# Autodesk Inventor assembly: Riser Base
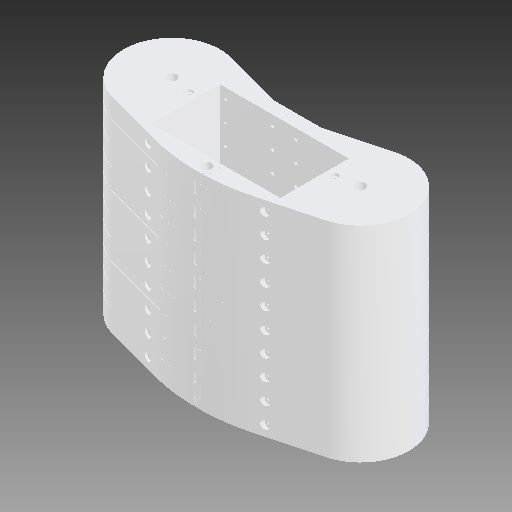
[picture p0: Inventor's stored thumbnail of the model, 512x512]
Saved by Autodesk Inventor 2017 SP1 (Build 210196100, 196)
## iProperties
Created: 2017-08-15
Part Number: Riser Base
Document SubType Name: Assembly
Designer: Zach
Author: Zach
## Documents named in this file (3)
- C:\Users\Zach\Documents\GitHub\cr-laundry-robot\src\Base\Rise Base Assembly\Riser Base.iam
- C:\Users\Zach\Documents\GitHub\cr-laundry-robot\src\Base\Rise Base Assembly\RB001.ipt
- C:\Users\Zach\Documents\GitHub\cr-laundry-robot\src\Base\Rise Base Assembly\RB002.ipt
## Components (40 placed, 2 different names)
1. RB001:1 — Mate:2, Mate:5, Mate:6, Mate:9, Mate:10, Mate:12, Mate:70
2. RB002:1 — Mate:1, Mate:9, Mate:10, Mate:69
3. RB001:2 — Mate:3, Mate:5, Mate:6, Mate:7, Mate:8, Mate:11, Mate:13
4. RB002:2 — Mate:4, Mate:7, Mate:8, Mate:68
5. RB001:3 — Mate:70, Mate:73
6. RB002:3 — Mate:69, Mate:72
7. RB001:4
8. RB002:4 — Mate:68, Mate:71
9. RB001:5 — Mate:79, Mate:82
10. RB002:5 — Mate:78, Mate:81
11. RB001:6
12. RB002:6 — Mate:77, Mate:80
13. RB001:7 — Mate:85, Mate:88
14. RB002:7 — Mate:84, Mate:87
15. RB001:8
16. RB002:8 — Mate:83, Mate:86
17. RB001:9 — Mate:91, Mate:94
18. RB002:9 — Mate:90, Mate:93
19. RB001:10
20. RB002:10 — Mate:89, Mate:92
21. RB001:11 — Mate:82, Mate:85
22. RB002:11 — Mate:81, Mate:84
23. RB001:12
24. RB002:12 — Mate:80, Mate:83
25. RB001:13 — Mate:88, Mate:91
26. RB002:13 — Mate:87, Mate:90
27. RB001:14
28. RB002:14 — Mate:86, Mate:89
29. RB001:15 — Mate:76, Mate:79
30. RB002:15 — Mate:75, Mate:78
31. RB001:16
32. RB002:16 — Mate:74, Mate:77
33. RB001:17 — Mate:94
34. RB002:17 — Mate:93
35. RB001:18
36. RB002:18 — Mate:92
37. RB001:19 — Mate:73, Mate:76
38. RB002:19 — Mate:72, Mate:75
39. RB001:20
40. RB002:20 — Mate:71, Mate:74
## Relationships (94: Mate 94)
- Mate:1: RB002:1
- Mate:2: RB001:1
- Mate:3: RB001:2
- Mate:4: RB002:2
- Mate:5: RB001:1 ↔ RB001:2
- Mate:6: RB001:1 ↔ RB001:2
- Mate:7: RB001:2 ↔ RB002:2
- Mate:8: RB001:2 ↔ RB002:2
- Mate:9: RB001:1 ↔ RB002:1
- Mate:10: RB001:1 ↔ RB002:1
- Mate:11: RB001:2
- Mate:12: RB001:1
- Mate:13: RB001:2
- [Mate]: RB001:3 ↔ RB001:4
- [Mate]: RB001:3 ↔ RB001:4
- [Mate]: RB001:4 ↔ RB002:4
- [Mate]: RB001:4 ↔ RB002:4
- [Mate]: RB001:3 ↔ RB002:3
- [Mate]: RB001:3 ↔ RB002:3
- [Mate]: RB001:5 ↔ RB001:6
- [Mate]: RB001:5 ↔ RB001:6
- [Mate]: RB001:6 ↔ RB002:6
- [Mate]: RB001:6 ↔ RB002:6
- [Mate]: RB001:5 ↔ RB002:5
- [Mate]: RB001:5 ↔ RB002:5
- [Mate]: RB001:7 ↔ RB001:8
- [Mate]: RB001:7 ↔ RB001:8
- [Mate]: RB001:8 ↔ RB002:8
- [Mate]: RB001:8 ↔ RB002:8
- [Mate]: RB001:7 ↔ RB002:7
- [Mate]: RB001:7 ↔ RB002:7
- [Mate]: RB001:9 ↔ RB001:10
- [Mate]: RB001:9 ↔ RB001:10
- [Mate]: RB001:10 ↔ RB002:10
- [Mate]: RB001:10 ↔ RB002:10
- [Mate]: RB001:9 ↔ RB002:9
- [Mate]: RB001:9 ↔ RB002:9
- [Mate]: RB001:11 ↔ RB001:12
- [Mate]: RB001:11 ↔ RB001:12
- [Mate]: RB001:12 ↔ RB002:12
- [Mate]: RB001:12 ↔ RB002:12
- [Mate]: RB001:11 ↔ RB002:11
- [Mate]: RB001:11 ↔ RB002:11
- [Mate]: RB001:13 ↔ RB001:14
- [Mate]: RB001:13 ↔ RB001:14
- [Mate]: RB001:14 ↔ RB002:14
- [Mate]: RB001:14 ↔ RB002:14
- [Mate]: RB001:13 ↔ RB002:13
- [Mate]: RB001:13 ↔ RB002:13
- [Mate]: RB001:15 ↔ RB001:16
- [Mate]: RB001:15 ↔ RB001:16
- [Mate]: RB001:16 ↔ RB002:16
- [Mate]: RB001:16 ↔ RB002:16
- [Mate]: RB001:15 ↔ RB002:15
- [Mate]: RB001:15 ↔ RB002:15
- [Mate]: RB001:17 ↔ RB001:18
- [Mate]: RB001:17 ↔ RB001:18
- [Mate]: RB001:18 ↔ RB002:18
- [Mate]: RB001:18 ↔ RB002:18
- [Mate]: RB001:17 ↔ RB002:17
- [Mate]: RB001:17 ↔ RB002:17
- [Mate]: RB001:19 ↔ RB001:20
- [Mate]: RB001:19 ↔ RB001:20
- [Mate]: RB001:20 ↔ RB002:20
- [Mate]: RB001:20 ↔ RB002:20
- [Mate]: RB001:19 ↔ RB002:19
- [Mate]: RB001:19 ↔ RB002:19
- Mate:68: RB002:2 ↔ RB002:4
- Mate:69: RB002:1 ↔ RB002:3
- Mate:70: RB001:1 ↔ RB001:3
- Mate:71: RB002:4 ↔ RB002:20
- Mate:72: RB002:3 ↔ RB002:19
- Mate:73: RB001:3 ↔ RB001:19
- Mate:74: RB002:16 ↔ RB002:20
- Mate:75: RB002:15 ↔ RB002:19
- Mate:76: RB001:15 ↔ RB001:19
- Mate:77: RB002:6 ↔ RB002:16
- Mate:78: RB002:5 ↔ RB002:15
- Mate:79: RB001:5 ↔ RB001:15
- Mate:80: RB002:6 ↔ RB002:12
- Mate:81: RB002:5 ↔ RB002:11
- Mate:82: RB001:5 ↔ RB001:11
- Mate:83: RB002:8 ↔ RB002:12
- Mate:84: RB002:7 ↔ RB002:11
- Mate:85: RB001:7 ↔ RB001:11
- Mate:86: RB002:8 ↔ RB002:14
- Mate:87: RB002:7 ↔ RB002:13
- Mate:88: RB001:7 ↔ RB001:13
- Mate:89: RB002:10 ↔ RB002:14
- Mate:90: RB002:9 ↔ RB002:13
- Mate:91: RB001:9 ↔ RB001:13
- Mate:92: RB002:10 ↔ RB002:18
- Mate:93: RB002:9 ↔ RB002:17
- Mate:94: RB001:9 ↔ RB001:17
## Named parameters: d13_d4 = 0 mm, d14_d5 = 0 mm, d15_d6 = 0 mm, d16_d7 = 0 mm, d17_d8 = 0 mm, d18_d9 = 0 mm, d19_d13_d4 = 0 mm, d20_d14_d5 = 0 mm, d21_d15_d6 = 0 mm, d22_d16_d7 = 0 mm, d23_d17_d8 = 0 mm, d24_d18_d9 = 0 mm, d25_d13_d4 = 0 mm, d26_d14_d5 = 0 mm, d27_d15_d6 = 0 mm, d28_d16_d7 = 0 mm, d29_d17_d8 = 0 mm, d30_d18_d9 = 0 mm, d31_d13_d4 = 0 mm, d32_d14_d5 = 0 mm, d33_d15_d6 = 0 mm, d34_d16_d7 = 0 mm, d35_d17_d8 = 0 mm, d36_d18_d9 = 0 mm, d37_d13_d4 = 0 mm, d38_d14_d5 = 0 mm, d39_d15_d6 = 0 mm, d40_d16_d7 = 0 mm, d41_d17_d8 = 0 mm, d42_d18_d9 = 0 mm, d43_d13_d4 = 0 mm, d44_d14_d5 = 0 mm, d45_d15_d6 = 0 mm, d46_d16_d7 = 0 mm, d47_d17_d8 = 0 mm, d48_d18_d9 = 0 mm, d49_d13_d4 = 0 mm, d50_d14_d5 = 0 mm, d51_d15_d6 = 0 mm, d52_d16_d7 = 0 mm, d53_d17_d8 = 0 mm, d54_d18_d9 = 0 mm, d55_d13_d4 = 0 mm, d56_d14_d5 = 0 mm, d57_d15_d6 = 0 mm, d58_d16_d7 = 0 mm, d59_d17_d8 = 0 mm, d60_d18_d9 = 0 mm, d61_d13_d4 = 0 mm, d62_d14_d5 = 0 mm, d63_d15_d6 = 0 mm, d64_d16_d7 = 0 mm, d65_d17_d8 = 0 mm, d66_d18_d9 = 0 mm
